# Autodesk Inventor assembly: idziemydalej
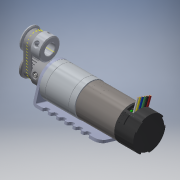
[picture p0: Inventor's stored thumbnail of the model, 180x180]
Saved by Autodesk Inventor 2019 (Build 230136000, 136)
## iProperties
Created: 2020-05-17
Part Number: idziemydalej
Document SubType Name: Assembly
Designer: estee
Author: estee
## Documents named in this file (10)
- C:\Users\estee\OneDrive\Pulpit\estere\1\MUM\projejt\idziemydalej.iam
- C:\Users\estee\OneDrive\Pulpit\estere\1\MUM\projejt\przekladnia.ipt
- C:\Users\estee\OneDrive\Pulpit\estere\1\MUM\projejt\zab.ipt
- C:\Users\estee\OneDrive\Pulpit\estere\1\MUM\projejt\pasek.ipt
- C:\Users\estee\OneDrive\Pulpit\estere\1\MUM\projejt\kolooooo.ipt
- C:\Users\estee\OneDrive\Pulpit\estere\1\MUM\projejt\kolo2\GT2_20T-sh8.ipt
- C:\Users\estee\OneDrive\Pulpit\estere\1\MUM\projejt\silnik25d-metal-gearmotor-378-499-encoder.ipt
- C:\Users\estee\OneDrive\Pulpit\estere\1\MUM\projejt\trzymakpololu-25d-mm-metal-gearmotor-bracket.ipt
- C:\Users\estee\OneDrive\Dokumenty\Inventor\Content Center Files\R2019\en-US\ISO 7045(2)\DIN EN ISO 7045 - M3 x 8 - 4.8 - Z.ipt
- C:\Users\estee\OneDrive\Dokumenty\Inventor\Content Center Files\R2019\en-US\ISO 4029\ISO 4029 - M3 x 6 - ISO.ipt
## Components (48 placed, 9 different names)
1. przekladnia:1 — Flush:1, Flush:2, Flush:3, Mate:1, Angle:1, Mate:2, Angle:2, Mate:3, Mate:4, Mate:5, Mate:7, Mate:9
2. pasek:1 — Mate:3, Mate:4, Mate:5
3. kolooooo:1 — Mate:6, Mate:7, Rotation:1, Mate:10, Mate:21, Mate:22, Mate:23
4. GT2_20T-sh8:1 — Mate:8, Mate:9, Rotation:1
5. silnik25d-metal-gearmotor-378-499-encoder:1 — Mate:10, Mate:11, Mate:12, Mate:13, Flush:5, Tangent:1
6. trzymakpololu-25d-mm-metal-gearmotor-bracket:1 — Mate:11, Mate:12, Mate:13, Mate:14, Mate:15, Mate:16, Mate:17, Mate:21
7. DIN EN ISO 7045 Z M3 x 8 - 4.8 - Z:1 — Mate:15, Mate:16
8. DIN EN ISO 7045 Z M3 x 8 - 4.8 - Z:2 — Mate:14, Mate:17
9. ISO 4029 M3 x 6:1 — Mate:23, Tangent:1
10. ISO 4029 M3 x 6:2 — Mate:22, Flush:5
11. zab:1 — Mate:1, Flush:4, Angle:1
12. zab:2
13. zab:3
14. zab:4
15. zab:5
16. zab:6
17. zab:7
18. zab:8
19. zab:9
20. zab:10
21. zab:11
22. zab:12
23. zab:13
24. zab:14
25. zab:15
26. zab:16
27. zab:17
28. zab:18
29. zab:19
30. zab:20
31. zab:21
32. zab:22
33. zab:23
34. zab:24
35. zab:25
36. zab:26
37. zab:27
38. zab:28
39. zab:29
40. zab:30
41. zab:31
42. zab:32
43. zab:33
44. zab:34
45. zab:35
46. zab:36
47. zab:37
48. zab:38
## Component patterns: (38 elements, first: zab:1)
## Relationships (29: Mate 20, Flush 5, Angle 2, RelateRotation 1, Tangent 1)
- Flush:1: przekladnia:1
- Flush:2: przekladnia:1
- Flush:3: przekladnia:1
- Mate:1: przekladnia:1 ↔ zab:1
- Flush:4 (-3 mm): zab:1
- Angle:1 (0 deg): przekladnia:1 ↔ zab:1
- Mate:2: przekladnia:1
- Angle:2 (0 deg): przekladnia:1
- Mate:3: przekladnia:1 ↔ pasek:1
- Mate:4: przekladnia:1 ↔ pasek:1
- Mate:5 (3 mm): przekladnia:1 ↔ pasek:1
- Mate:6: kolooooo:1
- Mate:7 (10.95 mm): przekladnia:1 ↔ kolooooo:1
- Mate:8: GT2_20T-sh8:1
- Mate:9 (10.95 mm): przekladnia:1 ↔ GT2_20T-sh8:1
- Rotation:1 [RelateRotation] (1 ul): kolooooo:1 ↔ GT2_20T-sh8:1
- Mate:10: kolooooo:1 ↔ silnik25d-metal-gearmotor-378-499-encoder:1
- Mate:11: silnik25d-metal-gearmotor-378-499-encoder:1 ↔ trzymakpololu-25d-mm-metal-gearmotor-bracket:1
- Mate:12: silnik25d-metal-gearmotor-378-499-encoder:1 ↔ trzymakpololu-25d-mm-metal-gearmotor-bracket:1
- Mate:13: silnik25d-metal-gearmotor-378-499-encoder:1 ↔ trzymakpololu-25d-mm-metal-gearmotor-bracket:1
- Mate:14: trzymakpololu-25d-mm-metal-gearmotor-bracket:1 ↔ DIN EN ISO 7045 Z M3 x 8 - 4.8 - Z:2
- Mate:15: trzymakpololu-25d-mm-metal-gearmotor-bracket:1 ↔ DIN EN ISO 7045 Z M3 x 8 - 4.8 - Z:1
- Mate:16: trzymakpololu-25d-mm-metal-gearmotor-bracket:1 ↔ DIN EN ISO 7045 Z M3 x 8 - 4.8 - Z:1
- Mate:17: trzymakpololu-25d-mm-metal-gearmotor-bracket:1 ↔ DIN EN ISO 7045 Z M3 x 8 - 4.8 - Z:2
- Mate:21 (2.5 mm): kolooooo:1 ↔ trzymakpololu-25d-mm-metal-gearmotor-bracket:1
- Mate:22: kolooooo:1 ↔ ISO 4029 M3 x 6:2
- Flush:5 (6 mm): silnik25d-metal-gearmotor-378-499-encoder:1 ↔ ISO 4029 M3 x 6:2
- Mate:23: kolooooo:1 ↔ ISO 4029 M3 x 6:1
- Tangent:1 (-10 mm): silnik25d-metal-gearmotor-378-499-encoder:1 ↔ ISO 4029 M3 x 6:1
